# Autodesk Inventor assembly: 200-ROCKER-BOGIE-ASM
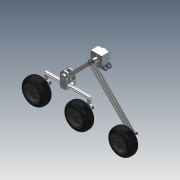
[picture p0: Inventor's stored thumbnail of the model, 180x180]
Saved by Autodesk Inventor 2018.2 (Build 222227000, 227)
## iProperties
Manager: feesmrt
Company: FRANC0R
Created: 2017-12-10
Part Number: 200-ROCKER-BOGIE-ASM
Material: Generisch
Document SubType Name: Assembly
Designer: feesmrt
Project: Rescue Robot
Description: Rocker Bogie Suspension
Engineer: feesmrt
Authority: feesmrt
Stock Number: 200-ROCKER-BOGIE-ASM
Author: feesmrt
Title: Rocker Bogie Suspension
Subject: Rescue Robot
Revision Number: 1
## Documents named in this file (4)
- D:\Programmierung\FRANC0R\CAD\02-Rocker-Bogie-Robot\200-ROCKER-BOGIE\200-ROCKER-BOGIE-ASM.iam
- D:\Programmierung\FRANC0R\CAD\02-Rocker-Bogie-Robot\200-ROCKER-BOGIE\200-ROCKER-ASM-01.iam
- D:\Programmierung\FRANC0R\CAD\02-Rocker-Bogie-Robot\200-ROCKER-BOGIE\200-BOGIE-ASM-01.iam
- D:\Programmierung\FRANC0R\CAD\02-Rocker-Bogie-Robot\200-ROCKER-BOGIE\200-50-WHEEL-CONNECTOR\200-50-WHEEL-CONNECTOR-ASM-01.iam
## Components (5 placed, 3 different names)
1. 200-ROCKER-ASM-01:1 [sub-assembly] — Passend:1, Passend:13, Passend:14, Passend:15, Passend:21, Fluchtend:2, Passend:22
2. 200-BOGIE-ASM-01:1 [sub-assembly] — Passend:1, Passend:13, Passend:14, Passend:15, Passend:16, Passend:17, Passend:18, Passend:19, Fluchtend:1, Passend:20
3. 200-50-WHEEL-CONNECTOR-ASM-01:1 [sub-assembly] — Passend:16, Passend:17, Passend:18
4. 200-50-WHEEL-CONNECTOR-ASM-01:2 [sub-assembly] — Passend:19, Fluchtend:1, Passend:20
5. 200-50-WHEEL-CONNECTOR-ASM-01:3 [sub-assembly] — Passend:21, Fluchtend:2, Passend:22
## Relationships (13: Mate 11, Flush 2)
- Passend:1 [Mate]: 200-ROCKER-ASM-01:1 ↔ 200-BOGIE-ASM-01:1
- Passend:13 [Mate]: 200-ROCKER-ASM-01:1 ↔ 200-BOGIE-ASM-01:1
- Passend:14 [Mate]: 200-ROCKER-ASM-01:1 ↔ 200-BOGIE-ASM-01:1
- Passend:15 [Mate]: 200-ROCKER-ASM-01:1 ↔ 200-BOGIE-ASM-01:1
- Passend:16 [Mate]: 200-BOGIE-ASM-01:1 ↔ 200-50-WHEEL-CONNECTOR-ASM-01:1
- Passend:17 [Mate]: 200-BOGIE-ASM-01:1 ↔ 200-50-WHEEL-CONNECTOR-ASM-01:1
- Passend:18 [Mate]: 200-BOGIE-ASM-01:1 ↔ 200-50-WHEEL-CONNECTOR-ASM-01:1
- Passend:19 [Mate]: 200-BOGIE-ASM-01:1 ↔ 200-50-WHEEL-CONNECTOR-ASM-01:2
- Fluchtend:1 [Flush]: 200-BOGIE-ASM-01:1 ↔ 200-50-WHEEL-CONNECTOR-ASM-01:2
- Passend:20 [Mate]: 200-BOGIE-ASM-01:1 ↔ 200-50-WHEEL-CONNECTOR-ASM-01:2
- Passend:21 [Mate]: 200-ROCKER-ASM-01:1 ↔ 200-50-WHEEL-CONNECTOR-ASM-01:3
- Fluchtend:2 [Flush]: 200-ROCKER-ASM-01:1 ↔ 200-50-WHEEL-CONNECTOR-ASM-01:3
- Passend:22 [Mate]: 200-ROCKER-ASM-01:1 ↔ 200-50-WHEEL-CONNECTOR-ASM-01:3
